# Autodesk Inventor assembly: s-assy-unit-j2
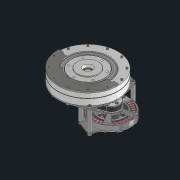
[picture p0: Inventor's stored thumbnail of the model, 180x180]
Saved by Autodesk Inventor 2022 (Build 260153000, 153)
## iProperties
Created: 2021-07-12
Part Number: s-assy-unit-j2
Document SubType Name: Assembly
Designer: yuta0
Mass: 876.37 g
Surface Area: 2474.15 cm^2
Volume: 379.417 cm^3
Density: 2.30978 g/cm^3
Author: yuta0
## Documents named in this file (11)
- C:\Users\yuta0\Documents\GitHub\catchrobo_hardware\assy-robot\s-assy-unit-j2.iam
- C:\Users\yuta0\Documents\GitHub\catchrobo_hardware\assy-robot\s-assy-unit-j2-2-gear.iam
- C:\Users\yuta0\Documents\GitHub\catchrobo_hardware\assy-robot\steel_plate2.ipt
- C:\Users\yuta0\Documents\GitHub\catchrobo_hardware\assy-robot\base41.ipt
- C:\Users\yuta0\Documents\GitHub\catchrobo_hardware\assy-robot\s-assy-motor.iam
- C:\Users\yuta0\Documents\GitHub\catchrobo_hardware\assy-robot\belt5.ipt
- C:\Users\yuta0\Documents\GitHub\catchrobo_hardware\assy-robot\s-assy-ring_gear-j2.iam
- C:\Users\yuta0\Documents\GitHub\catchrobo_hardware\assy-robot\ARF-430E.ipt
- C:\Users\yuta0\Documents\GitHub\catchrobo_hardware\assy-robot\base43.ipt
- C:\Users\yuta0\Documents\GitHub\catchrobo_hardware\assy-robot\CB4-6.ipt
- C:\Users\yuta0\Documents\GitHub\catchrobo_hardware\assy-shooter\MF126ZZ.ipt
## Components (10 placed, 10 different names)
1. s-assy-unit-j2-2-gear:1 [sub-assembly] — フラッシュ:1, メイト:52, メイト:53, メイト:57, メイト:58, メイト:59, メイト:77
2. s-assy-ring_gear-j2:1 [sub-assembly] — メイト:52, メイト:53, メイト:54, メイト:56, メイト:65, メイト:66, メイト:75
3. steel_plate2:1 — メイト:54, メイト:56, メイト:57
4. s-assy-motor:1 [sub-assembly] — メイト:65, メイト:66, メイト:70, メイト:72, メイト:74, メイト:75, メイト:78
5. base41:1 — メイト:58, メイト:59, メイト:62
6. belt5:1 — メイト:62, メイト:77, メイト:78
7. ARF-430E:1 — メイト:70, メイト:71, メイト:76
8. base43:1 — メイト:71, メイト:72
9. CB4-6:1 — メイト:74, メイト:76
10. MF126ZZ:1
## Relationships (19: Mate 18, Flush 1)
- フラッシュ:1 [Flush]: s-assy-unit-j2-2-gear:1
- メイト:52 [Mate]: s-assy-unit-j2-2-gear:1 ↔ s-assy-ring_gear-j2:1
- メイト:53 [Mate]: s-assy-unit-j2-2-gear:1 ↔ s-assy-ring_gear-j2:1
- メイト:54 [Mate]: s-assy-ring_gear-j2:1 ↔ steel_plate2:1
- メイト:56 [Mate]: s-assy-ring_gear-j2:1 ↔ steel_plate2:1
- メイト:57 [Mate]: s-assy-unit-j2-2-gear:1 ↔ steel_plate2:1
- メイト:58 [Mate]: s-assy-unit-j2-2-gear:1 ↔ base41:1
- メイト:59 [Mate]: s-assy-unit-j2-2-gear:1 ↔ base41:1
- メイト:62 [Mate] (0.5 mm): base41:1 ↔ belt5:1
- メイト:65 [Mate]: s-assy-ring_gear-j2:1 ↔ s-assy-motor:1
- メイト:66 [Mate]: s-assy-ring_gear-j2:1 ↔ s-assy-motor:1
- メイト:70 [Mate]: s-assy-motor:1 ↔ ARF-430E:1
- メイト:71 [Mate]: ARF-430E:1 ↔ base43:1
- メイト:72 [Mate]: s-assy-motor:1 ↔ base43:1
- メイト:74 [Mate]: s-assy-motor:1 ↔ CB4-6:1
- メイト:75 [Mate]: s-assy-ring_gear-j2:1 ↔ s-assy-motor:1
- メイト:76 [Mate]: ARF-430E:1 ↔ CB4-6:1
- メイト:77 [Mate]: s-assy-unit-j2-2-gear:1 ↔ belt5:1
- メイト:78 [Mate]: s-assy-motor:1 ↔ belt5:1
